# Autodesk Inventor assembly: AssamblyRobot
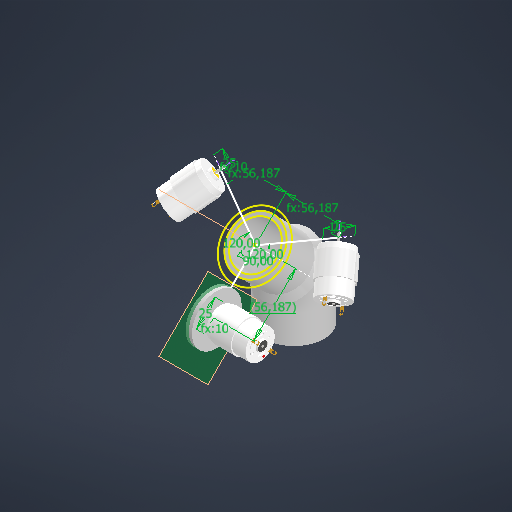
[picture p0: Inventor's stored thumbnail of the model, 512x512]
Saved by Autodesk Inventor 2026 (Build 300175050, 175E)
## iProperties
Created: 2025-07-17
Part Number: AssamblyRobot
Document SubType Name: Assembly
Designer: RubenPC
Author: RubenPC
## Documents named in this file (4)
- C:\Users\RubenPC\Code\RoboTT\AssamblyRobot.iam
- C:\Users\RubenPC\Code\RoboTT\assets\MABUCHI_MOTOR_385\MABUCHI_MOTOR_385\MABUCHI_MOTOR_385.ipt
- C:\Users\RubenPC\Code\RoboTT\assets\4880K691_Standard-Wall PVC Pipe Fitting for Water\4880K691_Standard-Wall PVC Pipe Fitting for Water\4880K691_Standard-Wall PVC Pipe Fitting for Water.ipt
- C:\Users\RubenPC\OneDrive\Documentos\Wheel.ipt
## Components (5 placed, 3 different names)
1. MABUCHI_MOTOR_385:1 — Mate:3, Mate:8
2. MABUCHI_MOTOR_385:2 — Mate:5, Mate:6
3. MABUCHI_MOTOR_385:3 — Mate:2, Mate:7
4. 4880K691_Standard-Wall PVC Pipe Fitting for Water:1 — Mate:1, Mate:2, Mate:3, Flush:1, Flush:2, Mate:5, Mate:6, Mate:7, Mate:8, Mate:9
5. Wheel:1 — Flush:3, Flush:4
## Relationships (13: Mate 9, Flush 4)
- Mate:1: 4880K691_Standard-Wall PVC Pipe Fitting for Water:1
- Mate:2: MABUCHI_MOTOR_385:3 ↔ 4880K691_Standard-Wall PVC Pipe Fitting for Water:1
- Mate:3: MABUCHI_MOTOR_385:1 ↔ 4880K691_Standard-Wall PVC Pipe Fitting for Water:1
- Flush:1: 4880K691_Standard-Wall PVC Pipe Fitting for Water:1
- Mate:4
- Flush:2: 4880K691_Standard-Wall PVC Pipe Fitting for Water:1
- Mate:5: MABUCHI_MOTOR_385:2 ↔ 4880K691_Standard-Wall PVC Pipe Fitting for Water:1
- Mate:6: MABUCHI_MOTOR_385:2 ↔ 4880K691_Standard-Wall PVC Pipe Fitting for Water:1
- Mate:7: MABUCHI_MOTOR_385:3 ↔ 4880K691_Standard-Wall PVC Pipe Fitting for Water:1
- Mate:8: MABUCHI_MOTOR_385:1 ↔ 4880K691_Standard-Wall PVC Pipe Fitting for Water:1
- Mate:9: 4880K691_Standard-Wall PVC Pipe Fitting for Water:1
- Flush:3: Wheel:1
- Flush:4: Wheel:1
